# Autodesk Inventor assembly: LCD+Case
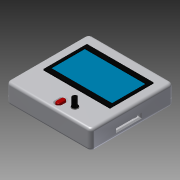
[picture p0: Inventor's stored thumbnail of the model, 180x180]
Saved by Autodesk Inventor 2015 SP1 (Build 190203100, 203)
## iProperties
Created: 2015-04-16
Part Number: LCD+Case
Document SubType Name: Assembly
Designer: Jack
Author: Jack
## Documents named in this file (6)
- C:\Users\Jack\ownCloud\Projects\CrossBot\InventorModel\Enclosure\LCDCase\LCD+Case.iam
- C:\Users\Jack\ownCloud\Projects\CrossBot\InventorModel\Electronics\LCD\GLCDKnockoff.ipt
- C:\Users\Jack\ownCloud\Projects\CrossBot\InventorModel\Enclosure\LCDCase\LCDDerivativeBottom1.ipt
- C:\Users\Jack\ownCloud\Projects\CrossBot\InventorModel\Enclosure\LCDCase\LCDDerivativeTop1.ipt
- C:\Users\Jack\ownCloud\Projects\CrossBot\InventorModel\Enclosure\LCDCase\LCDButton.ipt
- C:\Users\Jack\ownCloud\Projects\CrossBot\STLs\Enclosure\LCDEnclosure\LCDMount.ipt
## Components (5 placed, 5 different names)
1. GLCDKnockoff:1 — Mate:3, Mate:4, Mate:5, Mate:6, Mate:11, Mate:12, Mate:13, Mate:17, Mate:23
2. LCDDerivativeBottom1:1 — Mate:11, Mate:12, Mate:13, Mate:23
3. LCDDerivativeTop1:1 — Mate:3, Mate:4, Mate:5, Mate:6, Mate:14, Mate:17, Mate:18, Mate:20, Mate:21, Mate:22, Angle:1
4. LCDButton:1 — Mate:14, Mate:18, Angle:1
5. LCDMount:1 — Mate:20, Mate:21, Mate:22
## Relationships (15: Mate 14, Angle 1)
- Mate:3: GLCDKnockoff:1 ↔ LCDDerivativeTop1:1
- Mate:4: GLCDKnockoff:1 ↔ LCDDerivativeTop1:1
- Mate:5: GLCDKnockoff:1 ↔ LCDDerivativeTop1:1
- Mate:6: GLCDKnockoff:1 ↔ LCDDerivativeTop1:1
- Mate:11: GLCDKnockoff:1 ↔ LCDDerivativeBottom1:1
- Mate:12: GLCDKnockoff:1 ↔ LCDDerivativeBottom1:1
- Mate:13: GLCDKnockoff:1 ↔ LCDDerivativeBottom1:1
- Mate:14: LCDDerivativeTop1:1 ↔ LCDButton:1
- Mate:17: GLCDKnockoff:1 ↔ LCDDerivativeTop1:1
- Mate:18: LCDDerivativeTop1:1 ↔ LCDButton:1
- Mate:20: LCDDerivativeTop1:1 ↔ LCDMount:1
- Mate:21: LCDDerivativeTop1:1 ↔ LCDMount:1
- Mate:22: LCDDerivativeTop1:1 ↔ LCDMount:1
- Mate:23: GLCDKnockoff:1 ↔ LCDDerivativeBottom1:1
- Angle:1 (180 deg): LCDDerivativeTop1:1 ↔ LCDButton:1
